# Autodesk Inventor assembly: tension
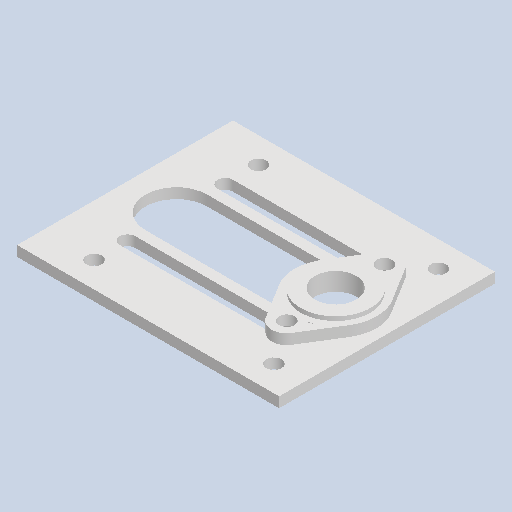
[picture p0: Inventor's stored thumbnail of the model, 512x512]
Saved by Autodesk Inventor 2025 (Build 290162000, 162)
## iProperties
Created: 2025-03-05
Part Number: tension
Document SubType Name: Assembly
Designer: Zhopa
Mass: 3.38203 g
Surface Area: 47.243 cm^2
Volume: 3.38203 cm^3
Density: 1 g/cm^3
Author: Zhopa
## Documents named in this file (4)
- C:\Users\onion\OneDrive - Kyushu University\共有用\工房共有ワンドライブ2024~2025用\ハード\NHK2025\Vova\elevator 3\subassemblies\tension.iam
- C:\Users\onion\OneDrive - Kyushu University\共有用\工房共有ワンドライブ2024~2025用\ハード\NHK2025\Vova\elevator 3\cnc\temsion1.ipt
- C:\Users\onion\OneDrive - Kyushu University\共有用\工房共有ワンドライブ2024~2025用\ハード\NHK2025\Vova\elevator 3\cnc\tension2.ipt
- C:\Users\onion\OneDrive - Kyushu University\共有用\工房共有ワンドライブ2024~2025用\ハード\NHK2025\Vova\elevator 3\bearings\DDLF-1280ZZ.ipt
## Components (3 placed, 3 different names)
1. temsion1:1 — 挿入:1, 挿入:2
2. tension2:1 — 挿入:1, 挿入:2, 挿入:3
3. DDLF-1280ZZ:1 — 挿入:3
## Relationships (3: Insert 3)
- 挿入:1 [Insert]: temsion1:1 ↔ tension2:1
- 挿入:2 [Insert]: temsion1:1 ↔ tension2:1
- 挿入:3 [Insert]: tension2:1 ↔ DDLF-1280ZZ:1
